# Autodesk Inventor assembly: ASY DMF 010 cap v2.1
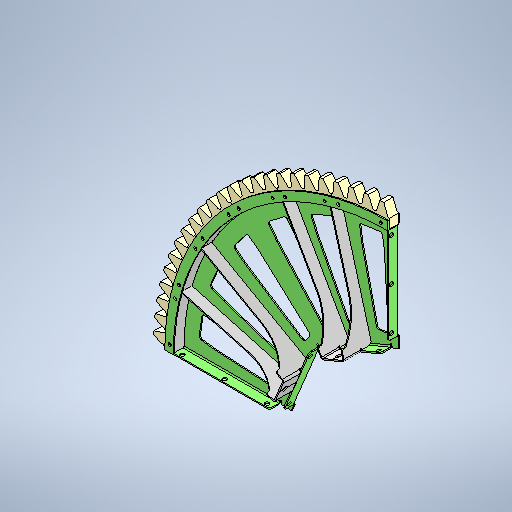
[picture p0: Inventor's stored thumbnail of the model, 512x512]
Saved by Autodesk Inventor 2026.2 (Build 302298010, 298A)
## iProperties
Created: 2024-04-30
Part Number: ASY DMF 010 cap v2.1
Document SubType Name: Assembly
Designer: admin
Author: admin
## Documents named in this file (7)
- C:\Users\admin\Documents\Inventor\DMF-Disk-Micro-Filter\Барабан v2.1\ASY DMF 010 cap v2.1.iam
- C:\Users\admin\Documents\Inventor\DMF-Disk-Micro-Filter\Барабан v2.1\DMF 2.1 01 43 Gear rim 3.ipt
- C:\Users\admin\Documents\Inventor\DMF-Disk-Micro-Filter\Барабан v2.1\DMF 2.1 01 44 Gear rim 4.ipt
- C:\Users\admin\Documents\Inventor\DMF-Disk-Micro-Filter\шестерни 06.09.2025\DMF sector big gear 2.1.ipt
- C:\Users\admin\Documents\Inventor\DMF-Disk-Micro-Filter\Барабан v2.1\DMF 2.1 Пластина паза большая.ipt
- C:\Users\admin\Documents\Inventor\DMF-Disk-Micro-Filter\Барабан v2.1\DMF 2.1 01 43 Gear rim 3_CPY.ipt
- C:\Users\admin\Documents\Inventor\DMF-Disk-Micro-Filter\Барабан v2.1\DMF 2.1 Пластина паза большая_MIR.ipt
## Components (13 placed, 7 different names)
1. DMF 2.1 01 43 Gear rim 3.ipt:2 — Flush:2, Flush:1, Flush:3, Mate:2, Flush:5, Mate:3, Flush:6, Flush:7, Mate:4
2. DMF 2.1 01 44 Gear rim 4.ipt:1 — Rigid:8
3. DMF sector big gear 2.1:6
4. DMF sector big gear 2.1:5
5. DMF sector big gear 2.1:4
6. DMF sector big gear 2.1:3
7. DMF sector big gear 2.1:2
8. DMF sector big gear 2.1.ipt:1
9. DMF 2.1 Пластина паза большая:2 — Mate:2, Flush:5, Rigid:9, Flush:7
10. DMF 2.1 01 43 Gear rim 3_CPY:1 — Rigid:8
11. DMF 2.1 Пластина паза большая_MIR:1 — Rigid:9
12. DMF 2.1 Пластина паза большая:3 — Mate:3, Flush:6, Mate:4
13. DMF 2.1 Пластина паза большая_MIR:2
## Relationships (18: WeldJoint 9, Flush 6, Mate 3)
- [WeldJoint]: DMF sector big gear 2.1:2 ↔ DMF sector big gear 2.1.ipt:1
- [WeldJoint]: DMF sector big gear 2.1:3 ↔ DMF sector big gear 2.1:2
- [WeldJoint]: DMF sector big gear 2.1:4 ↔ DMF sector big gear 2.1:3
- [WeldJoint]: DMF sector big gear 2.1:5 ↔ DMF sector big gear 2.1:4
- [WeldJoint]: DMF sector big gear 2.1:6 ↔ DMF sector big gear 2.1:5
- [WeldJoint]: DMF 2.1 01 43 Gear rim 3.ipt:2 ↔ DMF sector big gear 2.1.ipt:1
- Flush:2: DMF 2.1 01 43 Gear rim 3.ipt:2
- Flush:1: DMF 2.1 01 43 Gear rim 3.ipt:2
- Flush:3: DMF 2.1 01 43 Gear rim 3.ipt:2
- Mate:2: DMF 2.1 01 43 Gear rim 3.ipt:2 ↔ DMF 2.1 Пластина паза большая:2
- Flush:5: DMF 2.1 01 43 Gear rim 3.ipt:2 ↔ DMF 2.1 Пластина паза большая:2
- Rigid:8 [WeldJoint]: DMF 2.1 01 44 Gear rim 4.ipt:1 ↔ DMF 2.1 01 43 Gear rim 3_CPY:1
- Rigid:9 [WeldJoint]: DMF 2.1 Пластина паза большая:2 ↔ DMF 2.1 Пластина паза большая_MIR:1
- [WeldJoint]: DMF 2.1 Пластина паза большая:3 ↔ DMF 2.1 Пластина паза большая_MIR:2
- Mate:3: DMF 2.1 01 43 Gear rim 3.ipt:2 ↔ DMF 2.1 Пластина паза большая:3
- Flush:6: DMF 2.1 01 43 Gear rim 3.ipt:2 ↔ DMF 2.1 Пластина паза большая:3
- Flush:7: DMF 2.1 01 43 Gear rim 3.ipt:2 ↔ DMF 2.1 Пластина паза большая:2
- Mate:4: DMF 2.1 01 43 Gear rim 3.ipt:2 ↔ DMF 2.1 Пластина паза большая:3
## Named parameters: d63_d62 = 0 mm
